# Autodesk Inventor assembly: ENSAMBLAJE
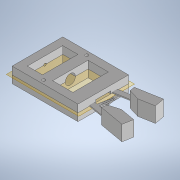
[picture p0: Inventor's stored thumbnail of the model, 180x180]
Saved by Autodesk Inventor 2022 (Build 260153000, 153)
## iProperties
Created: 2022-11-02
Part Number: ENSAMBLAJE
Document SubType Name: Assembly
Designer: Usuario
Author: Usuario
## Documents named in this file (5)
- C:\Users\Usuario\Documents\Cosas de Sebastian\Robotica\PROYECTO\CAD\GRIPPER\ENSAMBLAJE.iam
- C:\Users\Usuario\Documents\Cosas de Sebastian\Robotica\PROYECTO\CAD\GRIPPER\BASE.ipt
- C:\Users\Usuario\Documents\Cosas de Sebastian\Robotica\PROYECTO\CAD\GRIPPER\BASE_UP.ipt
- C:\Users\Usuario\Documents\Cosas de Sebastian\Robotica\PROYECTO\CAD\GRIPPER\PINZA_D.ipt
- C:\Users\Usuario\Documents\Cosas de Sebastian\Robotica\PROYECTO\CAD\GRIPPER\PINZA_I.ipt
## Components (4 placed, 4 different names)
1. BASE:1 — De rotación:1, De rotación:2, Rígido:1
2. BASE_UP:1 — Rígido:1
3. PINZA_D:1 — De rotación:1
4. PINZA_I:1 — De rotación:2
## Relationships (3: RevoluteJoint 2, WeldJoint 1)
- De rotación:1 [RevoluteJoint]: BASE:1 ↔ PINZA_D:1
- De rotación:2 [RevoluteJoint]: BASE:1 ↔ PINZA_I:1
- Rígido:1 [WeldJoint]: BASE:1 ↔ BASE_UP:1
